# Autodesk Inventor assembly: tester
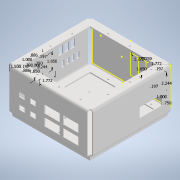
[picture p0: Inventor's stored thumbnail of the model, 180x180]
Saved by Autodesk Inventor 2020.2 (Build 242310000, 310)
## iProperties
Created: 2020-02-05
Part Number: tester
Document SubType Name: Assembly
Designer: ColinP
Author: ColinP
## Documents named in this file (11)
- C:\Users\ColinP\Documents\Inventor\HeaterControlIQC\sheetmetalversion\tester.iam
- C:\Users\ColinP\Documents\Inventor\HeaterControlIQC\sheetmetalversion\sheetmetalbottom.ipt
- C:\Users\ColinP\Documents\Inventor\HeaterControlIQC\sheetmetalversion\sheetmetalback.ipt
- C:\Users\ColinP\Documents\Inventor\HeaterControlIQC\sheetmetalversion\sheetmetalleftside.ipt
- C:\Users\ColinP\Documents\Inventor\HeaterControlIQC\sheetmetalversion\sheetmetalface.ipt
- C:\Users\ColinP\Documents\Inventor\HeaterControlIQC\sheetmetalversion\sheetmetalrightside.ipt
- C:\Users\ColinP\Documents\Inventor\HeaterControlIQC\sheetmetalversion\sheetmetallid.ipt
- C:\Users\ColinP\Documents\Inventor\HeaterControlIQC\CUI_VSK-S5-5UA-T (1)\CUI_VSK-S5-5UA-T.iam
- C:\Users\ColinP\Documents\Inventor\HeaterControlIQC\Qualtek_06AE2.ipt
- C:\Users\ColinP\Documents\Inventor\HeaterControlIQC\User Library-Thermocouple_Submini Jack.ipt
- C:\Users\ColinP\Documents\Inventor\HeaterControlIQC\4300-0705.ipt
## Components (15 placed, 10 different names)
1. sheetmetalbottom:1 — Mate:58, Mate:59, Mate:60
2. sheetmetalback:1 — Mate:4, Mate:7, Mate:10, Mate:11, Mate:30, Mate:31, Mate:45, Mate:57, Mate:60, Mate:61, Mate:62
3. sheetmetalface:1 — Mate:52, Mate:53, Mate:54, Mate:55, Mate:56
4. sheetmetalleftside:1 — Mate:4, Mate:7, Flush:1, Flush:2, Flush:3, Flush:4, Flush:5, Flush:6, Mate:33, Mate:34, Mate:35, Mate:36, Mate:37, Mate:38, Mate:39, Mate:40, Mate:41, Mate:42, Mate:43, Mate:44, Mate:54, Mate:58, Flush:7, Flush:8, Flush:9
5. sheetmetalrightside:1 — Mate:10, Mate:11, Mate:29, Mate:48, Mate:49, Mate:50, Mate:52, Mate:53, Mate:55, Mate:56, Mate:57, Mate:59
6. sheetmetallid:1 — Mate:29, Mate:30, Mate:31
7. CUI_VSK-S5-5UA-T:1 [sub-assembly] — Mate:45, Mate:61, Mate:62
8. Qualtek_06AE2:1 — Mate:48, Mate:49, Mate:50
9. User Library-Thermocouple_Submini Jack:1 — Mate:36, Mate:37, Mate:38
10. User Library-Thermocouple_Submini Jack:2 — Mate:39, Mate:40, Mate:41
11. User Library-Thermocouple_Submini Jack:3 — Mate:42, Mate:43, Mate:44
12. User Library-Thermocouple_Submini Jack:4 — Mate:33, Mate:34, Mate:35
13. 4300-0705:1 — Flush:4, Flush:5, Flush:6
14. 4300-0705:2 — Flush:7, Flush:8, Flush:9
15. 4300-0705:3 — Flush:1, Flush:2, Flush:3
## Relationships (43: Mate 34, Flush 9)
- Mate:4: sheetmetalback:1 ↔ sheetmetalleftside:1
- Mate:7: sheetmetalback:1 ↔ sheetmetalleftside:1
- Mate:10: sheetmetalback:1 ↔ sheetmetalrightside:1
- Mate:11: sheetmetalback:1 ↔ sheetmetalrightside:1
- Mate:29: sheetmetalrightside:1 ↔ sheetmetallid:1
- Mate:30: sheetmetalback:1 ↔ sheetmetallid:1
- Mate:31: sheetmetalback:1 ↔ sheetmetallid:1
- Flush:1: sheetmetalleftside:1 ↔ 4300-0705:3
- Flush:2: sheetmetalleftside:1 ↔ 4300-0705:3
- Flush:3: sheetmetalleftside:1 ↔ 4300-0705:3
- Flush:4: sheetmetalleftside:1 ↔ 4300-0705:1
- Flush:5: sheetmetalleftside:1 ↔ 4300-0705:1
- Flush:6: sheetmetalleftside:1 ↔ 4300-0705:1
- Mate:33: sheetmetalleftside:1 ↔ User Library-Thermocouple_Submini Jack:4
- Mate:34: sheetmetalleftside:1 ↔ User Library-Thermocouple_Submini Jack:4
- Mate:35: sheetmetalleftside:1 ↔ User Library-Thermocouple_Submini Jack:4
- Mate:36: sheetmetalleftside:1 ↔ User Library-Thermocouple_Submini Jack:1
- Mate:37: sheetmetalleftside:1 ↔ User Library-Thermocouple_Submini Jack:1
- Mate:38: sheetmetalleftside:1 ↔ User Library-Thermocouple_Submini Jack:1
- Mate:39: sheetmetalleftside:1 ↔ User Library-Thermocouple_Submini Jack:2
- Mate:40: sheetmetalleftside:1 ↔ User Library-Thermocouple_Submini Jack:2
- Mate:41: sheetmetalleftside:1 ↔ User Library-Thermocouple_Submini Jack:2
- Mate:42: sheetmetalleftside:1 ↔ User Library-Thermocouple_Submini Jack:3
- Mate:43: sheetmetalleftside:1 ↔ User Library-Thermocouple_Submini Jack:3
- Mate:44: sheetmetalleftside:1 ↔ User Library-Thermocouple_Submini Jack:3
- Mate:45: sheetmetalback:1 ↔ CUI_VSK-S5-5UA-T:1
- Mate:48: sheetmetalrightside:1 ↔ Qualtek_06AE2:1
- Mate:49: sheetmetalrightside:1 ↔ Qualtek_06AE2:1
- Mate:50: sheetmetalrightside:1 ↔ Qualtek_06AE2:1
- Mate:52: sheetmetalface:1 ↔ sheetmetalrightside:1
- Mate:53: sheetmetalface:1 ↔ sheetmetalrightside:1
- Mate:54: sheetmetalface:1 ↔ sheetmetalleftside:1
- Mate:55: sheetmetalface:1 ↔ sheetmetalrightside:1
- Mate:56: sheetmetalface:1 ↔ sheetmetalrightside:1
- Mate:57: sheetmetalback:1 ↔ sheetmetalrightside:1
- Mate:58: sheetmetalbottom:1 ↔ sheetmetalleftside:1
- Mate:59: sheetmetalbottom:1 ↔ sheetmetalrightside:1
- Mate:60: sheetmetalbottom:1 ↔ sheetmetalback:1
- Mate:61: sheetmetalback:1 ↔ CUI_VSK-S5-5UA-T:1
- Mate:62: sheetmetalback:1 ↔ CUI_VSK-S5-5UA-T:1
- Flush:7: sheetmetalleftside:1 ↔ 4300-0705:2
- Flush:8: sheetmetalleftside:1 ↔ 4300-0705:2
- Flush:9: sheetmetalleftside:1 ↔ 4300-0705:2
